# Autodesk Inventor assembly: Head
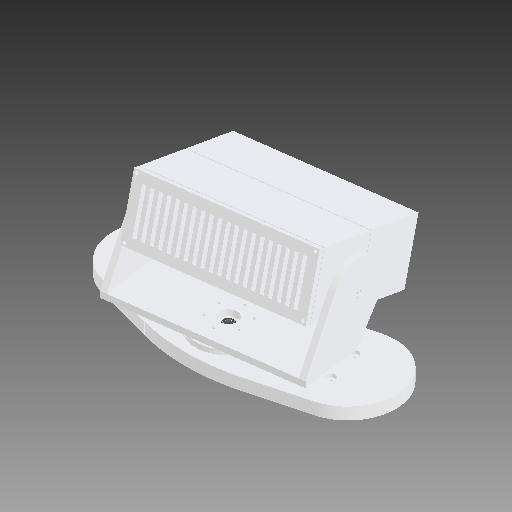
[picture p0: Inventor's stored thumbnail of the model, 512x512]
Saved by Autodesk Inventor 2017 SP1 (Build 210196100, 196)
## iProperties
Created: 2017-06-08
Part Number: Head
Document SubType Name: Assembly
Designer: zallen
Author: zallen
## Documents named in this file (14)
- C:\Users\Zach\Documents\GitHub\tr1\src\Head\Head.iam
- C:\Users\Zach\Documents\GitHub\tr1\src\Head\HA002.ipt
- C:\Users\Zach\Documents\GitHub\tr1\src\Head\HA004.ipt
- C:\Users\Zach\Documents\GitHub\tr1\src\Head\HA005.ipt
- C:\Users\Zach\Documents\GitHub\tr1\src\Head\HA006.ipt
- C:\Users\Zach\Documents\GitHub\tr1\lib\Xbox One Kinect\AS1.iam
- C:\Users\Zach\Documents\GitHub\tr1\src\Head\HA001.ipt
- C:\Users\Zach\Documents\GitHub\tr1\src\Head\HA007.ipt
- C:\Users\Zach\Documents\GitHub\tr1\lib\Strain Wave Gearbox\StrainWaveGearbox.iam
- C:\Users\Zach\Documents\GitHub\tr1\lib\DC Motor with Encoder\Motor.ipt
- C:\Users\Zach\Documents\GitHub\tr1\lib\4mm mounting hub.ipt
- C:\Users\Zach\Documents\GitHub\tr1\src\Head\HA009.ipt
- C:\Users\Zach\Documents\GitHub\tr1\src\Head\HA010.ipt
- C:\Users\Zach\Documents\GitHub\tr1\src\Head\HA011.ipt
## Components (17 placed, 13 different names)
1. HA001:1 — Mate:35, Mate:45, Mate:46, Mate:47, Mate:51, Mate:52, Mate:56, Mate:58, Mate:60
2. HA002:1 — Mate:1, Mate:9, Mate:26, Mate:27, Mate:28, Mate:29, Mate:30, Mate:42, Mate:43, Mate:44
3. HA004:1 — Mate:39, Mate:40, Mate:41, Mate:49, Mate:50, Mate:61, Mate:66, Mate:67
4. HA005:1 — Mate:17, Mate:19, Mate:53, Mate:54, Mate:55, Mate:57
5. HA006:1 — Mate:32, Mate:34, Flush:1, Mate:35, Mate:60
6. Kinect:1 [sub-assembly] — Mate:17, Mate:19, Mate:68
7. HA007:1 — Mate:26, Mate:27
8. HA007:2 — Mate:28, Mate:29, Mate:30
9. HA006:2 — Mate:32, Mate:34, Flush:1, Mate:59
10. StrainWaveGearbox:1 [sub-assembly] — Mate:39, Mate:40, Mate:41, Mate:42, Mate:43
11. Motor:1 — Mate:45, Mate:46, Mate:47, Mate:48, Mate:49
12. 4mm mounting hub:1 — Mate:48, Mate:50, Mate:51
13. HA009:1 — Mate:52, Mate:53, Mate:54, Mate:55, Mate:56, Mate:68
14. HA010:1 — Mate:57, Mate:58, Mate:59, Mate:63, Mate:64, Mate:65
15. Motor:2 — Mate:63, Mate:64, Mate:65
16. 4mm mounting hub:2 — Mate:61
17. HA011:1 — Mate:66, Mate:67
## Relationships (42: Mate 41, Flush 1)
- Mate:1: HA002:1
- Mate:9: HA002:1
- Mate:17: HA005:1 ↔ Kinect:1
- Mate:19: HA005:1 ↔ Kinect:1
- Mate:26: HA002:1 ↔ HA007:1
- Mate:27: HA002:1 ↔ HA007:1
- Mate:28: HA002:1 ↔ HA007:2
- Mate:29: HA002:1 ↔ HA007:2
- Mate:30: HA002:1 ↔ HA007:2
- Mate:32: HA006:1 ↔ HA006:2
- Mate:34: HA006:1 ↔ HA006:2
- Flush:1: HA006:1 ↔ HA006:2
- Mate:35: HA001:1 ↔ HA006:1
- Mate:39: HA004:1 ↔ StrainWaveGearbox:1
- Mate:40: HA004:1 ↔ StrainWaveGearbox:1
- Mate:41: HA004:1 ↔ StrainWaveGearbox:1
- Mate:42: HA002:1 ↔ StrainWaveGearbox:1
- Mate:43: HA002:1 ↔ StrainWaveGearbox:1
- Mate:44: HA002:1
- Mate:45: HA001:1 ↔ Motor:1
- Mate:46: HA001:1 ↔ Motor:1
- Mate:47: HA001:1 ↔ Motor:1
- Mate:48: Motor:1 ↔ 4mm mounting hub:1
- Mate:49: HA004:1 ↔ Motor:1
- Mate:50: HA004:1 ↔ 4mm mounting hub:1
- Mate:51: HA001:1 ↔ 4mm mounting hub:1
- Mate:52: HA001:1 ↔ HA009:1
- Mate:53: HA005:1 ↔ HA009:1
- Mate:54: HA005:1 ↔ HA009:1
- Mate:55: HA005:1 ↔ HA009:1
- Mate:56: HA001:1 ↔ HA009:1
- Mate:57: HA005:1 ↔ HA010:1
- Mate:58: HA001:1 ↔ HA010:1
- Mate:59: HA006:2 ↔ HA010:1
- Mate:60: HA001:1 ↔ HA006:1
- Mate:61: HA004:1 ↔ 4mm mounting hub:2
- Mate:63: HA010:1 ↔ Motor:2
- Mate:64: HA010:1 ↔ Motor:2
- Mate:65: HA010:1 ↔ Motor:2
- Mate:66: HA004:1 ↔ HA011:1
- Mate:67: HA004:1 ↔ HA011:1
- Mate:68: Kinect:1 ↔ HA009:1
